# Autodesk Inventor assembly: CollectorPrototype
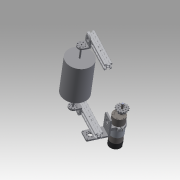
[picture p0: Inventor's stored thumbnail of the model, 180x180]
Saved by Autodesk Inventor 2016 (Build 200138000, 138)
## iProperties
Created: 2016-12-07
Part Number: CollectorPrototype
Document SubType Name: Assembly
Designer: Delta
Author: Delta
## Documents named in this file (12)
- C:\Robotics\CAD\2016-17_CAD\CollectorPrototype.iam
- C:\Robotics\CAD\COTSParts\Bosch Extrusion\Bosch 20x20 - 4.5 Part.Shoot.ipt
- C:\Robotics\CAD\2016-17_CAD\8InchAx.ipt
- C:\Robotics\CAD\2016-17_CAD\CollectorBrush.ipt
- C:\Robotics\CAD\COTSParts\Actobotics\615 parts\615102.ipt
- C:\Robotics\CAD\COTSParts\Actobotics\545 parts\545400.ipt
- C:\Robotics\CAD\COTSParts\Actobotics\545 parts\545576.ipt
- C:\Robotics\CAD\COTSParts\Actobotics\585 parts\585494.ipt
- C:\Robotics\CAD\COTSParts\Actobotics\am-3102NeveRest20 (1).ipt
- C:\Robotics\CAD\COTSParts\Actobotics\555 parts\555116.ipt
- C:\Robotics\CAD\COTSParts\Actobotics\535 parts\535216.ipt
- C:\Robotics\CAD\COTSParts\Bosch Extrusion\6mm block nut M4.ipt
## Components (21 placed, 11 different names)
1. 8InchAx:1 — Insert:3, Mate:1, Insert:7, Insert:8
2. CollectorBrush:1 — Insert:3, Mate:2
3. 615102:1 — Insert:4
4. 545400:1 — Mate:5, Mate:8, Mate:11, Mate:12, Mate:13, Mate:14
5. 545400:2 — Mate:6, Mate:7, Mate:30, Mate:31, Mate:32, Mate:33
6. 545576:1 — Insert:4, Mate:1, Mate:2
7. 545576:2 — Mate:37, Mate:38, Mate:39
8. 585494:1 — Mate:9, Mate:10, Mate:26, Mate:27, Mate:28, Mate:29
9. Bosch 20x20 - 4.5 Part.Shoot:1 — Mate:34, Mate:35, Mate:36, Flush:5, Flush:6
10. Bosch 20x20 - 4.5 Part.Shoot:2 — Mate:15, Mate:16, Mate:17, Mate:22, Mate:23, Mate:24, Mate:25, Flush:2, Flush:4, Flush:6
11. 615102:2 — Mate:39, Mate:40
12. am-3102NeveRest20 (1):1 — Insert:9, Mate:37, Mate:38, Mate:40
13. 555116:1 — Mate:9, Mate:10, Mate:29, Insert:9
14. 535216:1 — Mate:5, Insert:8, Mate:8
15. 535216:2 — Mate:6, Mate:7, Insert:7
16. 6mm block nut M4:1 — Mate:30, Mate:31, Mate:36, Flush:5
17. 6mm block nut M4:2 — Mate:24, Mate:25, Flush:2, Mate:27, Mate:28
18. 6mm block nut M4:3 — Mate:11, Mate:12, Mate:15, Mate:16
19. 6mm block nut M4:4 — Mate:13, Mate:14, Mate:17, Flush:4
20. 6mm block nut M4:5 — Mate:22, Mate:23, Mate:26
21. 6mm block nut M4:6 — Mate:32, Mate:33, Mate:34, Mate:35
## Relationships (43: Mate 34, Insert 5, Flush 4)
- Insert:3 (40.64 mm): 8InchAx:1 ↔ CollectorBrush:1
- Insert:4: 615102:1 ↔ 545576:1
- Mate:1: 8InchAx:1 ↔ 545576:1
- Mate:2: CollectorBrush:1 ↔ 545576:1
- Mate:5: 545400:1 ↔ 535216:1
- Mate:6: 545400:2 ↔ 535216:2
- Mate:7: 545400:2 ↔ 535216:2
- Insert:7: 8InchAx:1 ↔ 535216:2
- Insert:8: 8InchAx:1 ↔ 535216:1
- Mate:8: 545400:1 ↔ 535216:1
- Mate:9: 585494:1 ↔ 555116:1
- Mate:10: 585494:1 ↔ 555116:1
- Mate:11: 545400:1 ↔ 6mm block nut M4:3
- Mate:12: 545400:1 ↔ 6mm block nut M4:3
- Mate:13: 545400:1 ↔ 6mm block nut M4:4
- Mate:14: 545400:1 ↔ 6mm block nut M4:4
- Mate:15: Bosch 20x20 - 4.5 Part.Shoot:2 ↔ 6mm block nut M4:3
- Mate:16: Bosch 20x20 - 4.5 Part.Shoot:2 ↔ 6mm block nut M4:3
- Mate:17: Bosch 20x20 - 4.5 Part.Shoot:2 ↔ 6mm block nut M4:4
- Mate:22: Bosch 20x20 - 4.5 Part.Shoot:2 ↔ 6mm block nut M4:5
- Mate:23: Bosch 20x20 - 4.5 Part.Shoot:2 ↔ 6mm block nut M4:5
- Mate:24: Bosch 20x20 - 4.5 Part.Shoot:2 ↔ 6mm block nut M4:2
- Mate:25: Bosch 20x20 - 4.5 Part.Shoot:2 ↔ 6mm block nut M4:2
- Flush:2: Bosch 20x20 - 4.5 Part.Shoot:2 ↔ 6mm block nut M4:2
- Mate:26: 585494:1 ↔ 6mm block nut M4:5
- Mate:27: 585494:1 ↔ 6mm block nut M4:2
- Mate:28: 585494:1 ↔ 6mm block nut M4:2
- Mate:29: 585494:1 ↔ 555116:1
- Mate:30: 545400:2 ↔ 6mm block nut M4:1
- Mate:31: 545400:2 ↔ 6mm block nut M4:1
- Mate:32: 545400:2 ↔ 6mm block nut M4:6
- Mate:33: 545400:2 ↔ 6mm block nut M4:6
- Mate:34: Bosch 20x20 - 4.5 Part.Shoot:1 ↔ 6mm block nut M4:6
- Mate:35: Bosch 20x20 - 4.5 Part.Shoot:1 ↔ 6mm block nut M4:6
- Mate:36: Bosch 20x20 - 4.5 Part.Shoot:1 ↔ 6mm block nut M4:1
- Flush:4: Bosch 20x20 - 4.5 Part.Shoot:2 ↔ 6mm block nut M4:4
- Flush:5: Bosch 20x20 - 4.5 Part.Shoot:1 ↔ 6mm block nut M4:1
- Flush:6: Bosch 20x20 - 4.5 Part.Shoot:1 ↔ Bosch 20x20 - 4.5 Part.Shoot:2
- Insert:9: am-3102NeveRest20 (1):1 ↔ 555116:1
- Mate:37: 545576:2 ↔ am-3102NeveRest20 (1):1
- Mate:38: 545576:2 ↔ am-3102NeveRest20 (1):1
- Mate:39: 545576:2 ↔ 615102:2
- Mate:40: 615102:2 ↔ am-3102NeveRest20 (1):1
